# Autodesk Inventor assembly: #Spindexer
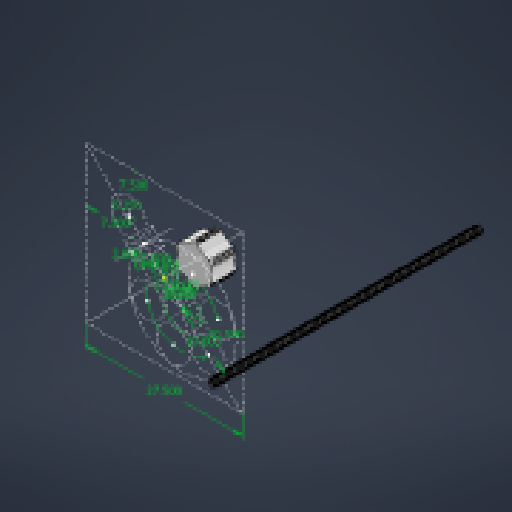
[picture p0: Inventor's stored thumbnail of the model, 512x512]
Saved by Autodesk Inventor 2026 (Build 300175000, 175)
## iProperties
Created: 2026-02-05
Part Number: #Spindexer
Document SubType Name: Assembly
Designer: Owen L
Author: Owen L
## Documents named in this file (5)
- C:\Users\littl\OneDrive\Documents\GitHub\2026-Robot-Mechanical\Spindexer\#Spindexer.iam
- C:\Users\littl\OneDrive\Documents\GitHub\2026-Robot-Mechanical\Spindexer\TEMP,BASE-SKETCH.ipt
- C:\Users\littl\OneDrive\Documents\GitHub\2026-Robot-Mechanical\Spindexer\3DPRINT,HUB.ipt
- C:\Users\littl\OneDrive\Documents\GitHub\2026-Robot-Mechanical\Spindexer\PURCHASED,MAXSPLINE,SPINDEXER,HUB.ipt
- C:\Users\littl\OneDrive\Documents\GitHub\2026-Robot-Mechanical\Spindexer\3DPRINT,HUB,CONE.ipt
## Components (4 placed, 4 different names)
1. TEMP,BASE-SKETCH:1
2. 3DPRINT,HUB:1 — Mate:9, Mate:10, Mate:11, Mate:12, Mate:13
3. PURCHASED,MAXSPLINE,SPINDEXER,HUB:1 — Mate:9, Mate:10, Mate:14
4. 3DPRINT,HUB,CONE:1 — Mate:11, Mate:12, Mate:13, Mate:14
## Relationships (6: Mate 6)
- Mate:9: 3DPRINT,HUB:1 ↔ PURCHASED,MAXSPLINE,SPINDEXER,HUB:1
- Mate:10: 3DPRINT,HUB:1 ↔ PURCHASED,MAXSPLINE,SPINDEXER,HUB:1
- Mate:11: 3DPRINT,HUB:1 ↔ 3DPRINT,HUB,CONE:1
- Mate:12: 3DPRINT,HUB:1 ↔ 3DPRINT,HUB,CONE:1
- Mate:13: 3DPRINT,HUB:1 ↔ 3DPRINT,HUB,CONE:1
- Mate:14: PURCHASED,MAXSPLINE,SPINDEXER,HUB:1 ↔ 3DPRINT,HUB,CONE:1
